# Autodesk Inventor assembly: Linear actuator
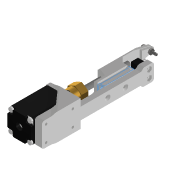
[picture p0: Inventor's stored thumbnail of the model, 180x180]
Saved by Autodesk Inventor 2020 (Build 240168000, 168)
## iProperties
Created: 2022-03-01
Part Number: Linear actuator
Document SubType Name: Assembly
Designer: ferrerx
Author: ferrerx
## Documents named in this file (13)
- C:\Users\ferrerx\Desktop\Projects\Elosegui lab\Cell stretcher\Linear actuator.iam
- C:\Users\ferrerx\Desktop\Projects\Elosegui lab\Cell stretcher\Motor holder.ipt
- C:\Users\ferrerx\Desktop\Projects\Elosegui lab\Cell stretcher\Nema 8.ipt
- C:\Users\ferrerx\Desktop\Projects\Elosegui lab\Cell stretcher\M4 threaded bar.ipt
- C:\Users\ferrerx\Desktop\Projects\Elosegui lab\Cell stretcher\Limit switch.ipt
- C:\Users\ferrerx\Desktop\Projects\Elosegui lab\Cell stretcher\Coupler.ipt
- C:\Users\ferrerx\Desktop\Projects\Elosegui lab\Cell stretcher\BSP10-25 bottom.iam
- C:\Users\ferrerx\Desktop\Projects\Elosegui lab\Cell stretcher\BSP10-25 top.iam
- C:\Users\ferrerx\Desktop\Projects\Elosegui lab\Cell stretcher\Nut holder.ipt
- C:\Users\ferrerx\Desktop\Projects\Elosegui lab\Cell stretcher\Clamp.ipt
- C:\Users\ferrerx\Documents\Inventor\Content Center Files\R2020\en-US\AS 1474(1)\AS 1474 - M2(1).ipt
- C:\Users\ferrerx\Documents\Inventor\Content Center Files\R2020\en-US\ANSI B18.3.1M(1)\ANSI B18.3.1M - M2x0.4 x 10(2).ipt
- C:\Users\ferrerx\Desktop\Projects\Elosegui lab\Cell stretcher\M4 nut.ipt
## Components (12 placed, 12 different names)
1. Motor holder:1 — Mate:1, Mate:2, Mate:3, Mate:14, Mate:15, Mate:16, Mate:17, Mate:18, Mate:19, Angle:1
2. Nema 8:1 — Mate:1, Mate:2, Mate:3, Mate:4, Mate:5, Mate:7
3. M4 threaded bar:1 — Mate:6, Mate:7, Mate:30
4. Limit switch:1 — Mate:14, Mate:15, Mate:16
5. Coupler:1 — Mate:4, Mate:5, Mate:6
6. BSP10-25 bottom:1 [sub-assembly] — Mate:17, Mate:18, Mate:19, Mate:20
7. BSP10-25 top:1 [sub-assembly] — Mate:20, Angle:1, Mate:21, Mate:22, Mate:23
8. Nut holder:1 — Mate:21, Mate:22, Mate:23, Mate:24, Flush:1, Mate:25, Mate:26, Mate:29, Mate:31
9. Clamp:1 — Mate:24, Flush:1, Mate:25, Mate:28
10. AS 1474 - Metric M2:1 — Mate:27, Mate:28
11. Broached Socket Head Cap Screw - Metric M2x0.4 x 10:1 — Mate:26, Mate:27, Mate:29
12. M4 nut:1 — Mate:30, Mate:31
## Relationships (27: Mate 25, Angle 1, Flush 1)
- Mate:1: Motor holder:1 ↔ Nema 8:1
- Mate:2: Motor holder:1 ↔ Nema 8:1
- Mate:3: Motor holder:1 ↔ Nema 8:1
- Mate:4: Nema 8:1 ↔ Coupler:1
- Mate:5 (0.5 mm): Nema 8:1 ↔ Coupler:1
- Mate:6: M4 threaded bar:1 ↔ Coupler:1
- Mate:7: Nema 8:1 ↔ M4 threaded bar:1
- Mate:14: Motor holder:1 ↔ Limit switch:1
- Mate:15: Motor holder:1 ↔ Limit switch:1
- Mate:16: Motor holder:1 ↔ Limit switch:1
- Mate:17: Motor holder:1 ↔ BSP10-25 bottom:1
- Mate:18: Motor holder:1 ↔ BSP10-25 bottom:1
- Mate:19: Motor holder:1 ↔ BSP10-25 bottom:1
- Mate:20: BSP10-25 bottom:1 ↔ BSP10-25 top:1
- Angle:1 (0 deg): Motor holder:1 ↔ BSP10-25 top:1
- Mate:21: BSP10-25 top:1 ↔ Nut holder:1
- Mate:22: BSP10-25 top:1 ↔ Nut holder:1
- Mate:23: BSP10-25 top:1 ↔ Nut holder:1
- Mate:24: Nut holder:1 ↔ Clamp:1
- Flush:1: Nut holder:1 ↔ Clamp:1
- Mate:25 (0.5 mm): Nut holder:1 ↔ Clamp:1
- Mate:26: Nut holder:1 ↔ Broached Socket Head Cap Screw - Metric M2x0.4 x 10:1
- Mate:27: AS 1474 - Metric M2:1 ↔ Broached Socket Head Cap Screw - Metric M2x0.4 x 10:1
- Mate:28: Clamp:1 ↔ AS 1474 - Metric M2:1
- Mate:29: Nut holder:1 ↔ Broached Socket Head Cap Screw - Metric M2x0.4 x 10:1
- Mate:30: M4 threaded bar:1 ↔ M4 nut:1
- Mate:31: Nut holder:1 ↔ M4 nut:1
